# Autodesk Inventor assembly: Assembly9
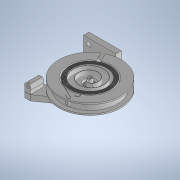
[picture p0: Inventor's stored thumbnail of the model, 180x180]
Saved by Autodesk Inventor 2022 (Build 260153070, 153G)
## iProperties
Created: 2022-03-06
Part Number: Assembly9
Document SubType Name: Assembly
Designer: a laptop
Author: a laptop
## Documents named in this file (10)
- C:\Users\a laptop\Desktop\MDL_2021_Project\Arm_Spool\Arm_Frame.iam
- C:\Users\a laptop\Desktop\MDL_2021_Project\Arm_Spool\Mount_Frame.ipt
- C:\Users\a laptop\Desktop\MDL_2021_Project\Return_Spool_Reel\Screws\M8 Washer98689A116_General Purpose 18-8 Stainless Steel Washer.ipt
- C:\Users\a laptop\Desktop\MDL_2021_Project\Return_Spool_Reel\Return_Spool_Mount\Design Accelerator\Bearing2.iam
- C:\Users\a laptop\Desktop\MDL_2021_Project\Return_Spool_Reel\SRM-12-06A.ipt
- C:\Users\a laptop\Desktop\MDL_2021_Project\Return_Spool_Reel\Bearing_Mount.ipt
- C:\Users\a laptop\Desktop\MDL_2021_Project\Return_Spool_Reel\Return_Spool.ipt
- C:\Users\a laptop\Desktop\MDL_2021_Project\Arm_Spool\Metal_Bushing.ipt
- C:\Users\a laptop\Desktop\MDL_2021_Project\Arm_Spool\Metal_Bushing_2.ipt
- C:\Users\a laptop\Desktop\MDL_2021_Project\Return_Spool_Reel\Springs\1842N11_Rotor Spring.ipt
## Components (9 placed, 9 different names)
1. Mount_Frame:1 — Mate:1, Mate:2, Mate:3, Mate:4, Mate:10, Mate:12, Mate:13, Mate:14
2. M8 Washer98689A116_General Purpose 18-8 Stainless Steel Washer:1 — Mate:7, Mate:8, Mate:9
3. Bearing:1 [sub-assembly] — Mate:9, Mate:5, Mate:11, Flush:1, Mate:17
4. SRM-12-06A:1 — Mate:1, Mate:2, Mate:3, Mate:6
5. Bearing_Mount:1 — Mate:4, Mate:6, Mate:7, Mate:8, Mate:5, Mate:10, Mate:16, Angle:1
6. Return_Spool:1 — Mate:11, Flush:1
7. Metal_Bushing:1 — Mate:12, Mate:13, Mate:14, Mate:15, Flush:2
8. Metal_Bushing_2:1 — Mate:15, Flush:2
9. 1842N11_Rotor Spring:1 — Mate:16, Mate:17, Angle:1
## Relationships (20: Mate 17, Flush 2, Angle 1)
- Mate:1: Mount_Frame:1 ↔ SRM-12-06A:1
- Mate:2: Mount_Frame:1 ↔ SRM-12-06A:1
- Mate:3: Mount_Frame:1 ↔ SRM-12-06A:1
- Mate:4: Mount_Frame:1 ↔ Bearing_Mount:1
- Mate:5: Bearing:1 ↔ Bearing_Mount:1
- Mate:6: SRM-12-06A:1 ↔ Bearing_Mount:1
- Mate:7: M8 Washer98689A116_General Purpose 18-8 Stainless Steel Washer:1 ↔ Bearing_Mount:1
- Mate:8: M8 Washer98689A116_General Purpose 18-8 Stainless Steel Washer:1 ↔ Bearing_Mount:1
- Mate:9: M8 Washer98689A116_General Purpose 18-8 Stainless Steel Washer:1 ↔ Bearing:1
- Mate:10: Mount_Frame:1 ↔ Bearing_Mount:1
- Mate:11: Bearing:1 ↔ Return_Spool:1
- Flush:1: Bearing:1 ↔ Return_Spool:1
- Mate:12: Mount_Frame:1 ↔ Metal_Bushing:1
- Mate:13: Mount_Frame:1 ↔ Metal_Bushing:1
- Mate:14: Mount_Frame:1 ↔ Metal_Bushing:1
- Mate:15: Metal_Bushing:1 ↔ Metal_Bushing_2:1
- Flush:2: Metal_Bushing:1 ↔ Metal_Bushing_2:1
- Mate:16: Bearing_Mount:1 ↔ 1842N11_Rotor Spring:1
- Mate:17: Bearing:1 ↔ 1842N11_Rotor Spring:1
- Angle:1 (0 deg): Bearing_Mount:1 ↔ 1842N11_Rotor Spring:1
